# Autodesk Inventor assembly: Robot
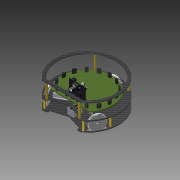
[picture p0: Inventor's stored thumbnail of the model, 180x180]
Saved by Autodesk Inventor 2015 (Build 190159000, 159)
## iProperties
Created: 2016-08-02
Part Number: Robot
Document SubType Name: Assembly
Designer: James Yelland
Author: James Yelland
## Documents named in this file (13)
- C:\Users\James Yelland\git\Layers-2017\Models\Robot.iam
- C:\Users\James Yelland\git\Layers-2017\Models\Bottom Plate.ipt
- C:\Users\James Yelland\git\Layers-2017\Models\Motor Mount.ipt
- C:\Users\James Yelland\git\Layers-2017\Models\Standoff 30.ipt
- C:\Users\James Yelland\git\Layers-2017\Models\Motor.ipt
- C:\Users\James Yelland\git\Layers-2017\Models\Wheel.ipt
- C:\Users\James Yelland\git\Layers-2017\Models\Middle Plate.ipt
- C:\Users\James Yelland\git\Layers-2017\Models\PCB.ipt
- C:\Users\James Yelland\git\Layers-2017\Models\Standoff 10.ipt
- C:\Users\James Yelland\git\Layers-2017\Models\Imported Components\Pixy(CMUcam5)\Pixy(CMUcam5).iam
- C:\Users\James Yelland\git\Layers-2017\Models\Solenoid.ipt
- C:\Users\James Yelland\git\Layers-2017\Models\Standoff 50.ipt
- C:\Users\James Yelland\git\Layers-2017\Models\Handle Ring.ipt
## Components (28 placed, 12 different names)
1. Bottom Plate:1 — Mate:1, Mate:2, Mate:3, Mate:4, Mate:5, Mate:6, Mate:7, Mate:8, Mate:9, Mate:10, Mate:11, Mate:12, Mate:13, Mate:14, Mate:15, Mate:16, Mate:17, Mate:18, Mate:19, Mate:20, Mate:21, Mate:57, Mate:59
2. Motor Mount:1 — Mate:1, Mate:2, Mate:6, Mate:24, Mate:25, Mate:26
3. Motor Mount:2 — Mate:3, Mate:4, Mate:5, Mate:23, Mate:27, Mate:28
4. Motor Mount:3 — Mate:7, Mate:8, Mate:9, Mate:22, Mate:29, Mate:30
5. Standoff 30:1 — Mate:20, Mate:21, Mate:35
6. Standoff 30:2 — Mate:18, Mate:19, Mate:34
7. Standoff 30:3 — Mate:16, Mate:17
8. Standoff 30:4 — Mate:14, Mate:15
9. Standoff 30:5 — Mate:12, Mate:13, Mate:36
10. Standoff 30:6 — Mate:10, Mate:11
11. Motor:1 — Mate:24, Mate:25, Mate:26, Mate:33, Flush:3
12. Motor:2 — Mate:23, Mate:27, Mate:28, Mate:31, Flush:1
13. Motor:3 — Mate:22, Mate:29, Mate:30, Mate:32, Flush:2
14. Wheel:1 — Mate:33, Flush:3
15. Wheel:2 — Mate:32, Flush:2
16. Wheel:3 — Mate:31, Flush:1
17. Middle Plate:1 — Mate:34, Mate:35, Mate:36, Mate:37, Mate:38, Mate:39, Mate:40, Mate:41, Mate:42, Mate:60, Mate:61, Mate:62, Mate:63, Mate:64, Mate:65, Mate:66, Mate:67
18. PCB:1 — Mate:43, Mate:44, Mate:45, Mate:58, Flush:4
19. Standoff 10:1 — Mate:39, Mate:40, Mate:43
20. Standoff 10:2 — Mate:38, Mate:41, Mate:44
21. Standoff 10:3 — Mate:37, Mate:42, Mate:45
22. Pixy(CMUcam5):1 [sub-assembly] — Mate:57, Mate:58
23. Solenoid:1 — Mate:59, Flush:4
24. Standoff 50:1 — Mate:63, Mate:64
25. Standoff 50:2 — Mate:62, Mate:66, Mate:69
26. Standoff 50:3 — Mate:61, Mate:67, Mate:68, Mate:70
27. Standoff 50:4 — Mate:60, Mate:65
28. Handle Ring:1 — Mate:68, Mate:69, Mate:70
## Relationships (63: Mate 59, Flush 4)
- Mate:1: Bottom Plate:1 ↔ Motor Mount:1
- Mate:2: Bottom Plate:1 ↔ Motor Mount:1
- Mate:3: Bottom Plate:1 ↔ Motor Mount:2
- Mate:4: Bottom Plate:1 ↔ Motor Mount:2
- Mate:5: Bottom Plate:1 ↔ Motor Mount:2
- Mate:6: Bottom Plate:1 ↔ Motor Mount:1
- Mate:7: Bottom Plate:1 ↔ Motor Mount:3
- Mate:8: Bottom Plate:1 ↔ Motor Mount:3
- Mate:9: Bottom Plate:1 ↔ Motor Mount:3
- Mate:10: Bottom Plate:1 ↔ Standoff 30:6
- Mate:11: Bottom Plate:1 ↔ Standoff 30:6
- Mate:12: Bottom Plate:1 ↔ Standoff 30:5
- Mate:13: Bottom Plate:1 ↔ Standoff 30:5
- Mate:14: Bottom Plate:1 ↔ Standoff 30:4
- Mate:15: Bottom Plate:1 ↔ Standoff 30:4
- Mate:16: Bottom Plate:1 ↔ Standoff 30:3
- Mate:17: Bottom Plate:1 ↔ Standoff 30:3
- Mate:18: Bottom Plate:1 ↔ Standoff 30:2
- Mate:19: Bottom Plate:1 ↔ Standoff 30:2
- Mate:20: Bottom Plate:1 ↔ Standoff 30:1
- Mate:21: Bottom Plate:1 ↔ Standoff 30:1
- Mate:22: Motor Mount:3 ↔ Motor:3
- Mate:23: Motor Mount:2 ↔ Motor:2
- Mate:24: Motor Mount:1 ↔ Motor:1
- Mate:25: Motor Mount:1 ↔ Motor:1
- Mate:26: Motor Mount:1 ↔ Motor:1
- Mate:27: Motor Mount:2 ↔ Motor:2
- Mate:28: Motor Mount:2 ↔ Motor:2
- Mate:29: Motor Mount:3 ↔ Motor:3
- Mate:30: Motor Mount:3 ↔ Motor:3
- Mate:31: Motor:2 ↔ Wheel:3
- Flush:1 (3 mm): Motor:2 ↔ Wheel:3
- Mate:32: Motor:3 ↔ Wheel:2
- Flush:2 (-3 mm): Motor:3 ↔ Wheel:2
- Mate:33: Motor:1 ↔ Wheel:1
- Flush:3 (-3 mm): Motor:1 ↔ Wheel:1
- Mate:34: Standoff 30:2 ↔ Middle Plate:1
- Mate:35: Standoff 30:1 ↔ Middle Plate:1
- Mate:36: Standoff 30:5 ↔ Middle Plate:1
- Mate:37: Middle Plate:1 ↔ Standoff 10:3
- Mate:38: Middle Plate:1 ↔ Standoff 10:2
- Mate:39: Middle Plate:1 ↔ Standoff 10:1
- Mate:40: Middle Plate:1 ↔ Standoff 10:1
- Mate:41: Middle Plate:1 ↔ Standoff 10:2
- Mate:42: Middle Plate:1 ↔ Standoff 10:3
- Mate:43: PCB:1 ↔ Standoff 10:1
- Mate:44: PCB:1 ↔ Standoff 10:2
- Mate:45: PCB:1 ↔ Standoff 10:3
- Mate:57 (33 mm): Bottom Plate:1 ↔ Pixy(CMUcam5):1
- Mate:58 (3 mm): PCB:1 ↔ Pixy(CMUcam5):1
- Mate:59: Bottom Plate:1 ↔ Solenoid:1
- Flush:4: PCB:1 ↔ Solenoid:1
- Mate:60: Middle Plate:1 ↔ Standoff 50:4
- Mate:61: Middle Plate:1 ↔ Standoff 50:3
- Mate:62: Middle Plate:1 ↔ Standoff 50:2
- Mate:63: Middle Plate:1 ↔ Standoff 50:1
- Mate:64: Middle Plate:1 ↔ Standoff 50:1
- Mate:65: Middle Plate:1 ↔ Standoff 50:4
- Mate:66: Middle Plate:1 ↔ Standoff 50:2
- Mate:67: Middle Plate:1 ↔ Standoff 50:3
- Mate:68: Standoff 50:3 ↔ Handle Ring:1
- Mate:69: Standoff 50:2 ↔ Handle Ring:1
- Mate:70: Standoff 50:3 ↔ Handle Ring:1
